# Autodesk Inventor assembly: DHS-3239
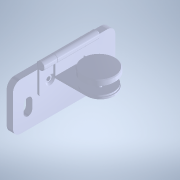
[picture p0: Inventor's stored thumbnail of the model, 180x180]
Saved by Autodesk Inventor 2021 (Build 250183000, 183)
## iProperties
Created: 2018-09-18
Part Number: DHS-3239
Document SubType Name: Assembly
Designer: gisen
Sending System: Autodesk Inventor 2014
Preprocessor: ST-DEVELOPER v15.2
Title: C:\Users\AMS43\Documents\Inventor\AMS\未_次回差し替え用_stp\DHS-3239.stp
Author: AMS43
## Documents named in this file (8)
- D:\GitProjects\CAD-Data\GeneralComponentsTemplate\Hinges\Hinge-DHS-3239.iam
- D:\GitProjects\CAD-Data\GeneralComponentsTemplate\Hinges\Hinge-DHS-3239\DHS-3239_本体.ipt
- D:\GitProjects\CAD-Data\GeneralComponentsTemplate\Hinges\Hinge-DHS-3239\DHS-3239_アーム.ipt
- D:\GitProjects\CAD-Data\GeneralComponentsTemplate\Hinges\Hinge-DHS-3239\DHS-3239_スピンヘッド.ipt
- D:\GitProjects\CAD-Data\GeneralComponentsTemplate\Hinges\Hinge-DHS-3239\DHS-3239_トラスねじ.ipt
- D:\GitProjects\CAD-Data\GeneralComponentsTemplate\Hinges\Hinge-DHS-3239\DHS-3239_ワッシャー.ipt
- D:\GitProjects\CAD-Data\GeneralComponentsTemplate\Hinges\Hinge-DHS-3239\DHS-3239_軸.ipt
- D:\GitProjects\CAD-Data\GeneralComponentsTemplate\Hinges\Hinge-DHS-3239\DHS-3239_プレート.ipt
## Components (8 placed, 7 different names)
1. DHS-3239_本体:1 — メイト:5, メイト:11, メイト:12, メイト:13, メイト:14, メイト:15
2. DHS-3239_アーム:1 — メイト:2, メイト:4, メイト:9, メイト:10, メイト:11
3. DHS-3239_スピンヘッド:1 — メイト:6, メイト:7, メイト:8, メイト:16
4. DHS-3239_トラスねじ:1 — メイト:8, メイト:9, メイト:10
5. DHS-3239_ワッシャー:1 — メイト:1, メイト:3, メイト:6, メイト:7
6. DHS-3239_軸:1 — メイト:4, メイト:5, メイト:15
7. DHS-3239_ワッシャー:2 — メイト:1, メイト:2, メイト:3
8. DHS-3239_プレート:1 — メイト:12, メイト:13, メイト:14
## Relationships (16: Mate 16)
- メイト:1 [Mate] (5 mm): DHS-3239_ワッシャー:1 ↔ DHS-3239_ワッシャー:2
- メイト:2 [Mate]: DHS-3239_アーム:1 ↔ DHS-3239_ワッシャー:2
- メイト:3 [Mate]: DHS-3239_ワッシャー:1 ↔ DHS-3239_ワッシャー:2
- メイト:4 [Mate]: DHS-3239_アーム:1 ↔ DHS-3239_軸:1
- メイト:5 [Mate]: DHS-3239_本体:1 ↔ DHS-3239_軸:1
- メイト:6 [Mate]: DHS-3239_スピンヘッド:1 ↔ DHS-3239_ワッシャー:1
- メイト:7 [Mate]: DHS-3239_スピンヘッド:1 ↔ DHS-3239_ワッシャー:1
- メイト:8 [Mate]: DHS-3239_スピンヘッド:1 ↔ DHS-3239_トラスねじ:1
- メイト:9 [Mate]: DHS-3239_アーム:1 ↔ DHS-3239_トラスねじ:1
- メイト:10 [Mate]: DHS-3239_アーム:1 ↔ DHS-3239_トラスねじ:1
- メイト:11 [Mate]: DHS-3239_本体:1 ↔ DHS-3239_アーム:1
- メイト:12 [Mate]: DHS-3239_本体:1 ↔ DHS-3239_プレート:1
- メイト:13 [Mate]: DHS-3239_本体:1 ↔ DHS-3239_プレート:1
- メイト:14 [Mate]: DHS-3239_本体:1 ↔ DHS-3239_プレート:1
- メイト:15 [Mate]: DHS-3239_本体:1 ↔ DHS-3239_軸:1
- メイト:16 [Mate]: DHS-3239_スピンヘッド:1
